# Autodesk Inventor assembly: printer
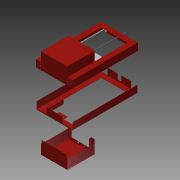
[picture p0: Inventor's stored thumbnail of the model, 180x180]
Saved by Autodesk Inventor 2014 SP2 (Build 180246200, 246)
## iProperties
Created: 2016-09-18
Part Number: printer
Document SubType Name: Assembly
Designer: cruiser
Mass: 4053.89 g
Surface Area: 12776.7 cm^2
Volume: 846.542 cm^3
Density: 4.78877 g/cm^3
Author: cruiser
## Documents named in this file (15)
- C:\Users\cruiser\Desktop\models\3d printers\laserresin5\printer.iam
- C:\Users\cruiser\Desktop\models\3d printers\laserresin5\frame_front.ipt
- C:\Users\cruiser\Desktop\models\3d printers\laserresin5\frame_back.ipt
- C:\Users\cruiser\Desktop\models\3d printers\laserresin5\drawer.ipt
- C:\Users\cruiser\Desktop\models\3d printers\laserresin5\reservoir.ipt
- C:\Users\cruiser\Desktop\models\3d printers\laserresin5\tray.ipt
- C:\Users\cruiser\Desktop\models\3d printers\laserresin5\crane.ipt
- C:\Users\cruiser\Desktop\models\3d printers\laserresin5\platform.ipt
- C:\Users\cruiser\Desktop\models\3d printers\laserresin5\handle.ipt
- C:\Users\cruiser\Desktop\models\3d printers\laserresin5\laserholder.ipt
- C:\Users\cruiser\Desktop\models\3d printers\laserresin5\nema17.ipt
- C:\Users\cruiser\Desktop\models\3d printers\laserresin5\lmk8luu.ipt
- C:\Users\cruiser\Desktop\models\3d printers\laserresin5\threaded_rod.ipt
- C:\Users\cruiser\Desktop\models\3d printers\laserresin5\shf8.ipt
- C:\Users\cruiser\Desktop\models\3d printers\laserresin5\m8_rail.ipt
## Components (21 placed, 14 different names)
1. frame_front:1 — Flush:1, Flush:2, Mate:1, Mate:2, Mate:8, Mate:9, Mate:10, Mate:17, Mate:19, Mate:22, Mate:26, Mate:38, Mate:39, Mate:40, Mate:41, Mate:42, Mate:43, Mate:44, Mate:45, Mate:46, Mate:47, Mate:48, Mate:49, Flush:7, Flush:8
2. frame_back:1 — Flush:1, Flush:2, Mate:11, Mate:18, Mate:22
3. drawer:1 — Mate:1, Mate:10, Mate:19, Mate:23, Mate:24, Mate:26
4. drawer:2 — Mate:2, Mate:11, Mate:25
5. reservoir:1 — Mate:5, Flush:4, Mate:13, Mate:14, Mate:15, Mate:16, Mate:23, Mate:24, Mate:25, Flush:6
6. tray:1 — Mate:5, Flush:4, Flush:6
7. crane:1 — Mate:6, Flush:5, Mate:8, Mate:9, Mate:27, Mate:28, Mate:29, Mate:30, Mate:31, Mate:32, Mate:33, Mate:34, Mate:35
8. platform:1 — Mate:6, Flush:5
9. handle:1 — Mate:13, Mate:14
10. handle:2 — Mate:15, Mate:16
11. laserholder:1 — Mate:17, Mate:18
12. nema17:1 — Mate:27, Mate:28, Mate:29, Mate:36, Mate:37
13. lmk8luu:1 — Mate:30, Mate:34, Mate:35
14. lmk8luu:2 — Mate:31, Mate:32, Mate:33
15. threaded_rod:1 — Mate:36, Mate:37
16. shf8:1 — Mate:44, Mate:45, Mate:46
17. shf8:2 — Mate:41, Mate:42, Mate:43
18. shf8:3 — Mate:47, Mate:48, Mate:49, Mate:51
19. shf8:4 — Mate:38, Mate:39, Mate:40, Mate:50
20. m8_rail:1 — Mate:50, Flush:7
21. m8_rail:2 — Mate:51, Flush:8
## Relationships (52: Mate 45, Flush 7)
- Flush:1: frame_front:1 ↔ frame_back:1
- Flush:2: frame_front:1 ↔ frame_back:1
- Mate:1: frame_front:1 ↔ drawer:1
- Mate:2: frame_front:1 ↔ drawer:2
- Mate:5: reservoir:1 ↔ tray:1
- Flush:4: reservoir:1 ↔ tray:1
- Mate:6: crane:1 ↔ platform:1
- Flush:5: crane:1 ↔ platform:1
- Mate:8: frame_front:1 ↔ crane:1
- Mate:9: frame_front:1 ↔ crane:1
- Mate:10: frame_front:1 ↔ drawer:1
- Mate:11: frame_back:1 ↔ drawer:2
- Mate:13: reservoir:1 ↔ handle:1
- Mate:14: reservoir:1 ↔ handle:1
- Mate:15: reservoir:1 ↔ handle:2
- Mate:16: reservoir:1 ↔ handle:2
- Mate:17: frame_front:1 ↔ laserholder:1
- Mate:18: frame_back:1 ↔ laserholder:1
- Mate:19: frame_front:1 ↔ drawer:1
- Mate:22: frame_front:1 ↔ frame_back:1
- Mate:23: drawer:1 ↔ reservoir:1
- Mate:24: drawer:1 ↔ reservoir:1
- Mate:25: drawer:2 ↔ reservoir:1
- Flush:6: reservoir:1 ↔ tray:1
- Mate:26: frame_front:1 ↔ drawer:1
- Mate:27: crane:1 ↔ nema17:1
- Mate:28: crane:1 ↔ nema17:1
- Mate:29: crane:1 ↔ nema17:1
- Mate:30: crane:1 ↔ lmk8luu:1
- Mate:31: crane:1 ↔ lmk8luu:2
- Mate:32: crane:1 ↔ lmk8luu:2
- Mate:33: crane:1 ↔ lmk8luu:2
- Mate:34: crane:1 ↔ lmk8luu:1
- Mate:35: crane:1 ↔ lmk8luu:1
- Mate:36: nema17:1 ↔ threaded_rod:1
- Mate:37: nema17:1 ↔ threaded_rod:1
- Mate:38: frame_front:1 ↔ shf8:4
- Mate:39: frame_front:1 ↔ shf8:4
- Mate:40: frame_front:1 ↔ shf8:4
- Mate:41: frame_front:1 ↔ shf8:2
- Mate:42: frame_front:1 ↔ shf8:2
- Mate:43: frame_front:1 ↔ shf8:2
- Mate:44: frame_front:1 ↔ shf8:1
- Mate:45: frame_front:1 ↔ shf8:1
- Mate:46: frame_front:1 ↔ shf8:1
- Mate:47: frame_front:1 ↔ shf8:3
- Mate:48: frame_front:1 ↔ shf8:3
- Mate:49: frame_front:1 ↔ shf8:3
- Mate:50: shf8:4 ↔ m8_rail:1
- Flush:7: frame_front:1 ↔ m8_rail:1
- Mate:51: shf8:3 ↔ m8_rail:2
- Flush:8: frame_front:1 ↔ m8_rail:2
